# Autodesk Inventor assembly: main
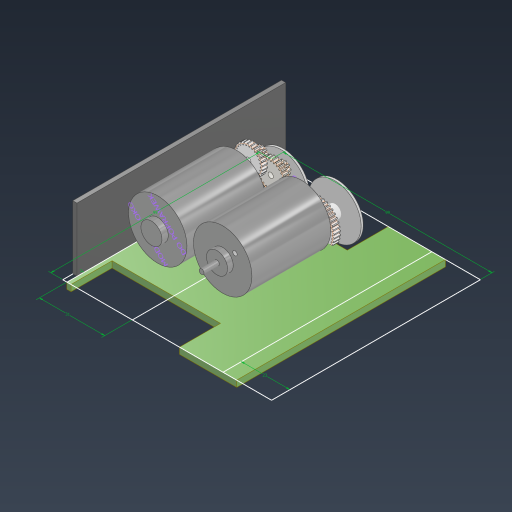
[picture p0: Inventor's stored thumbnail of the model, 512x512]
Saved by Autodesk Inventor 2023 (Build 270158000, 158)
## iProperties
Created: 2025-03-29
Part Number: main
Document SubType Name: Assembly
Designer: szymo
Mass: 421.477 g
Surface Area: 797.238 cm^2
Volume: 148.723 cm^3
Density: 2.83398 g/cm^3
Author: szymo
## Documents named in this file (25)
- D:\tech\robotyka\robots\evangelion\inventor-project\main.iam
- D:\tech\robotyka\robots\evangelion\inventor-project\base.ipt
- D:\tech\robotyka\robots\evangelion\inventor-project\Sensor LUNA.ipt
- D:\tech\robotyka\robots\evangelion\inventor-project\lipo-3s-550mah.ipt
- D:\tech\robotyka\robots\evangelion\inventor-project\tattu450_3s.ipt
- D:\tech\robotyka\robots\evangelion\inventor-project\oponka-dziurawa-prototyp\rs385.ipt
- D:\tech\robotyka\robots\evangelion\inventor-project\oponka-dziurawa-prototyp\back.ipt
- D:\tech\robotyka\robots\evangelion\inventor-project\Gears\Design Accelerator\Przekładnia walcowa14.ipt
- D:\tech\robotyka\robots\evangelion\inventor-project\Gears\Design Accelerator\Przekładnia walcowa22.ipt
- D:\tech\robotyka\robots\evangelion\inventor-project\Gears\Design Accelerator\Przekładnia walcowa23.ipt
- D:\tech\robotyka\robots\evangelion\inventor-project\Gears\Design Accelerator\Przekładnia walcowa24.ipt
- D:\tech\robotyka\robots\evangelion\inventor-project\Gears\Design Accelerator\Przekładnia walcowa12.ipt
- D:\tech\robotyka\robots\evangelion\inventor-project\Gears\Design Accelerator\Przekładnia walcowa13.ipt
- D:\tech\robotyka\robots\evangelion\inventor-project\oponka-dziurawa-prototyp\wheel.ipt
- D:\tech\robotyka\robots\evangelion\inventor-project\Lozysko GFM-0608-2.ipt
- D:\tech\robotyka\robots\evangelion\inventor-project\tattu450_2s.ipt
- D:\tech\robotyka\robots\evangelion\inventor-project\oponka-dziurawa-prototyp\front-mechanizm.iam
- D:\tech\robotyka\robots\evangelion\inventor-project\tfminis\LiDAR Benewake TFMini.iam
- D:\tech\robotyka\robots\evangelion\inventor-project\128x32-OLED.ipt
- D:\tech\robotyka\robots\evangelion\inventor-project\interface_board.ipt
- D:\tech\robotyka\robots\evangelion\inventor-project\front.iam
- D:\tech\robotyka\robots\evangelion\inventor-project\side-right.ipt
- D:\tech\robotyka\robots\evangelion\inventor-project\oponka-dziurawa-prototyp\front-mechanizm_MIR.iam
- D:\tech\robotyka\robots\evangelion\inventor-project\Lozysko GFM-0608-06 very shorted.ipt
- D:\tech\robotyka\robots\evangelion\inventor-project\Lozysko HK0608.ipt
## Components (44 placed, 20 different names)
1. base:1 — Mate:5, Mate:6, Mate:7, Flush:10, Flush:11, Mate:63, Mate:64, Tangent:24, Mate:65, Flush:16, Flush:17, Flush:18, Flush:19, Angle:4, Angle:5, Angle:6, Mate:101, Mate:102, Angle:7
2. rs385:2 — Tangent:6, Mate:53, Mate:54, Tangent:21, Tangent:22, Tangent:23, Mate:101, Tangent:34
3. rs385:3 — Tangent:4, Tangent:5, Mate:102
4. Sensor LUNA:1 — Mate:62, Mate:64, Flush:14
5. Sensor LUNA:2 — Mate:61, Mate:63, Flush:13
6. lipo-3s-550mah:1
7. tattu450_3s:1 — Tangent:21
8. back:1 — Mate:5, Mate:6, Tangent:4, Mate:7, Tangent:5, Tangent:6, Angle:2, Flush:9, Flush:12, Tangent:28, Angle:4
9. tattu450_2s:1 — Flush:9, Mate:58, Tangent:22, Flush:10, Flush:13, Flush:14
10. tattu450_2s:2 — Mate:58, Tangent:23, Mate:61, Mate:62, Flush:11
11. front-mechanizm:1 [sub-assembly] — Tangent:24, Mate:65
12. front-mechanizm_MIR:1 [sub-assembly]
13. front:1 [sub-assembly]
14. side-right:1 — Flush:16, Flush:17, Flush:18, Flush:19
15. LiDAR Benewake TFMini:1 [sub-assembly]
16. LiDAR Benewake TFMini:2 [sub-assembly]
17. 128x32-OLED:1
18. interface_board:1
19. Lozysko HK0608:1 — Mate:91, Mate:93
20. Lozysko HK0608:2 — Mate:92, Mate:94, Tangent:34
21. Przekładnia walcowa2:10 — Tangent:32
22. Przekładnia walcowa1:8 — Mate:99, Mate:100, Tangent:33
23. Przekładnia walcowa1:3
24. Przekładnia walcowa2:1 — Tangent:33
25. Przekładnia walcowa1:2 — Mate:99
26. Przekładnia walcowa1:7 — Tangent:30, Tangent:31
27. Przekładnia walcowa2:9 — Mate:95, Mate:96, Mate:100, Tangent:32
28. Przekładnia walcowa2:4 — Angle:6, Mate:92, Mate:94, Mate:95, Tangent:30, Mate:103, Angle:7
29. Przekładnia walcowa2:3 — Angle:5, Mate:91, Mate:93, Mate:96, Tangent:31, Mate:103
30. wheel:1 — Tangent:29, Flush:20
31. wheel:2 — Tangent:28, Tangent:29, Flush:20
32. Lozysko GFM-0608-06 very shorted:2 — Mate:81, Mate:83
33. Lozysko GFM-0608-06 very shorted:1 — Mate:80, Mate:82
34. Przekładnia walcowa1:4
35. Przekładnia walcowa2:5 — Tangent:17
36. Przekładnia walcowa2:6
37. Przekładnia walcowa2:7 — Mate:55, Angle:3, Mate:80, Mate:82
38. Przekładnia walcowa1:5
39. Przekładnia walcowa1:6 — Mate:53, Mate:54
40. Przekładnia walcowa2:8 — Tangent:17, Mate:55, Mate:81, Mate:83
41. wheel:3 — Tangent:25
42. wheel:4 — Tangent:25
43. Lozysko GFM-0608-2:3
44. Lozysko GFM-0608-2:4
## Relationships (102: Mate 50, Tangent 21, Flush 18, Angle 7, RelateRotation 6)
- [Angle] (0 deg): base:1 ↔ rs385:3
- [Tangent]: rs385:2 ↔ rs385:3
- [Mate]: rs385:3 ↔ Przekładnia walcowa1:3
- [Mate] (0.5 mm): rs385:3 ↔ Przekładnia walcowa1:3
- Mate:5: base:1 ↔ back:1
- Mate:6: base:1 ↔ back:1
- Tangent:4: rs385:3 ↔ back:1
- Mate:7: base:1 ↔ back:1
- Tangent:5: rs385:3 ↔ back:1
- Tangent:6: rs385:2 ↔ back:1
- [Tangent]: Przekładnia walcowa1:3 ↔ Przekładnia walcowa1:2
- [Flush]: Przekładnia walcowa1:3 ↔ Przekładnia walcowa1:2
- [Mate]: Przekładnia walcowa2:1 ↔ Przekładnia walcowa1:2
- [Mate]: Przekładnia walcowa2:1 ↔ Przekładnia walcowa1:2
- [Mate]: Przekładnia walcowa2:4 ↔ wheel:1
- [Flush] (1 mm): Przekładnia walcowa2:4 ↔ wheel:1
- [Mate]: Przekładnia walcowa2:3 ↔ wheel:2
- [Flush] (1 mm): Przekładnia walcowa2:3 ↔ wheel:2
- Angle:2 (0 deg): back:1
- Flush:5 (-49.5 mm)
- [Tangent]: Przekładnia walcowa1:5 ↔ Przekładnia walcowa1:6
- [RelateRotation] (0.4 ul): Przekładnia walcowa1:5 ↔ Przekładnia walcowa1:6
- [Flush]: Przekładnia walcowa1:5 ↔ Przekładnia walcowa1:6
- [Mate]: Przekładnia walcowa2:5 ↔ Przekładnia walcowa1:5
- [Mate]: Przekładnia walcowa2:5 ↔ Przekładnia walcowa1:5
- [RelateRotation] (1 ul): Przekładnia walcowa2:5 ↔ Przekładnia walcowa1:5
- [Mate] (0.1 mm): Przekładnia walcowa2:6 ↔ Przekładnia walcowa1:5
- [Tangent]: Przekładnia walcowa2:5 ↔ Przekładnia walcowa2:6
- [RelateRotation] (0.333 ul): Przekładnia walcowa2:5 ↔ Przekładnia walcowa2:6
- [Mate]: Przekładnia walcowa1:4 ↔ Przekładnia walcowa2:6
- [Mate]: Przekładnia walcowa1:4 ↔ Przekładnia walcowa2:6
- [RelateRotation] (0.5 ul): Przekładnia walcowa1:4 ↔ Przekładnia walcowa2:6
- [Mate] (0.1 mm): Przekładnia walcowa2:6 ↔ Przekładnia walcowa2:7
- [RelateRotation] (0.375 ul): Przekładnia walcowa1:4 ↔ Przekładnia walcowa2:7
- [Mate] (0.1 mm): Przekładnia walcowa2:6 ↔ Przekładnia walcowa2:8
- [Tangent]: Przekładnia walcowa1:4 ↔ Przekładnia walcowa2:8
- [RelateRotation] (2.667 ul): Przekładnia walcowa1:4 ↔ Przekładnia walcowa2:8
- [Mate]: Przekładnia walcowa2:8 ↔ wheel:3
- [Flush] (1 mm): Przekładnia walcowa2:8 ↔ wheel:3
- [Mate]: Przekładnia walcowa2:7 ↔ wheel:4
- [Flush] (1 mm): Przekładnia walcowa2:7 ↔ wheel:4
- [Mate]: Przekładnia walcowa2:7 ↔ Lozysko GFM-0608-2:4
- [Mate]: Przekładnia walcowa2:7 ↔ Lozysko GFM-0608-2:4
- [Mate]: Przekładnia walcowa2:8 ↔ Lozysko GFM-0608-2:3
- [Mate]: Przekładnia walcowa2:8 ↔ Lozysko GFM-0608-2:3
- Mate:53 (0.5 mm): rs385:2 ↔ Przekładnia walcowa1:6
- Mate:54: rs385:2 ↔ Przekładnia walcowa1:6
- Tangent:17 (0.5 mm): Przekładnia walcowa2:5 ↔ Przekładnia walcowa2:8
- Mate:55: Przekładnia walcowa2:7 ↔ Przekładnia walcowa2:8
- Angle:3 (0 deg): Przekładnia walcowa2:7
- Tangent:21 (1 mm): rs385:2 ↔ tattu450_3s:1
- Flush:9: back:1 ↔ tattu450_2s:1
- Mate:58: tattu450_2s:1 ↔ tattu450_2s:2
- Tangent:22: rs385:2 ↔ tattu450_2s:1
- Tangent:23: rs385:2 ↔ tattu450_2s:2
- Mate:61: Sensor LUNA:2 ↔ tattu450_2s:2
- Mate:62: Sensor LUNA:1 ↔ tattu450_2s:2
- Flush:10 (15.5 mm): base:1 ↔ tattu450_2s:1
- Flush:11 (15.5 mm): base:1 ↔ tattu450_2s:2
- Mate:63 (1.5 mm): base:1 ↔ Sensor LUNA:2
- Mate:64 (1.5 mm): base:1 ↔ Sensor LUNA:1
- Flush:12 (87 mm): back:1
- Tangent:24 (3.5 mm): base:1 ↔ front-mechanizm:1
- Mate:65: base:1 ↔ front-mechanizm:1
- Flush:13: Sensor LUNA:2 ↔ tattu450_2s:1
- Flush:14: Sensor LUNA:1 ↔ tattu450_2s:1
- Tangent:25 (1 mm): wheel:3 ↔ wheel:4
- Flush:16: base:1 ↔ side-right:1
- Flush:17: base:1 ↔ side-right:1
- Flush:18: base:1 ↔ side-right:1
- Flush:19: base:1 ↔ side-right:1
- Mate:80 (0.1 mm): Lozysko GFM-0608-06 very shorted:1 ↔ Przekładnia walcowa2:7
- Mate:81 (0.1 mm): Lozysko GFM-0608-06 very shorted:2 ↔ Przekładnia walcowa2:8
- Mate:82: Lozysko GFM-0608-06 very shorted:1 ↔ Przekładnia walcowa2:7
- Mate:83: Lozysko GFM-0608-06 very shorted:2 ↔ Przekładnia walcowa2:8
- [Mate]: Przekładnia walcowa1:7 ↔ Przekładnia walcowa2:9
- [Mate]: Przekładnia walcowa1:7 ↔ Przekładnia walcowa2:9
- Tangent:28 (0.5 mm): back:1 ↔ wheel:2
- Angle:4 (-90 deg): base:1 ↔ back:1
- Tangent:29 (0.5 mm): wheel:1 ↔ wheel:2
- Angle:5 (180 deg): base:1 ↔ Przekładnia walcowa2:3
- Angle:6 (180 deg): base:1 ↔ Przekładnia walcowa2:4
- Flush:20: wheel:1 ↔ wheel:2
- Mate:91: Lozysko HK0608:1 ↔ Przekładnia walcowa2:3
- Mate:92: Lozysko HK0608:2 ↔ Przekładnia walcowa2:4
- Mate:93 (0.1 mm): Lozysko HK0608:1 ↔ Przekładnia walcowa2:3
- Mate:94 (0.1 mm): Lozysko HK0608:2 ↔ Przekładnia walcowa2:4
- Mate:95 (0.1 mm): Przekładnia walcowa2:9 ↔ Przekładnia walcowa2:4
- Mate:96 (0.1 mm): Przekładnia walcowa2:9 ↔ Przekładnia walcowa2:3
- Tangent:30: Przekładnia walcowa1:7 ↔ Przekładnia walcowa2:4
- Tangent:31: Przekładnia walcowa1:7 ↔ Przekładnia walcowa2:3
- [Mate]: Przekładnia walcowa2:10 ↔ Przekładnia walcowa1:8
- [Mate]: Przekładnia walcowa2:10 ↔ Przekładnia walcowa1:8
- Mate:99 (0.1 mm): Przekładnia walcowa1:8 ↔ Przekładnia walcowa1:2
- Mate:100 (0.1 mm): Przekładnia walcowa1:8 ↔ Przekładnia walcowa2:9
- Tangent:32: Przekładnia walcowa2:10 ↔ Przekładnia walcowa2:9
- Tangent:33: Przekładnia walcowa1:8 ↔ Przekładnia walcowa2:1
- Mate:101 (29.65 mm): base:1 ↔ rs385:2
- Mate:102 (29.65 mm): base:1 ↔ rs385:3
- Mate:103: Przekładnia walcowa2:4 ↔ Przekładnia walcowa2:3
- Angle:7 (0 deg): base:1 ↔ Przekładnia walcowa2:4
- Tangent:34 (0.2 mm): rs385:2 ↔ Lozysko HK0608:2
## Named parameters: d53_d28 = 0 mm, d54_d29 = 0 mm, d208_d31 = 0.1 mm, d209_d32 = 0 mm, d210_d58_d33 = 0.333, d211_d59_d34 = 0 mm, d212_d60_d35 = 0 mm, d213_d61_d36 = 0.5, d214_d62_d37 = 0.1 mm, d216_d64_d39 = 0.375, d217_d67 = 1 mm, d218_d61 = 0.1 mm, d219_d62 = 0 mm, d220_d63 = 2.667, d221_d64 = 0 mm, d222_d65 = 1 mm, d223_d66 = 0 mm, d230_d88 = 0 mm, d231_d89 = 0 mm, d232_d90 = 0 mm, d233_d91 = 0 mm, d234_d25 = 0 mm, d235_d26 = 0.4, d236_d27 = 0 mm, d237_d53_d28 = 0 mm, d238_d54_d29 = 0 mm, d239_d30 = 1, d333_d59_d34 = 0 mm, d334_d60_d35 = 0 mm, d357_d53_d28 = 0 mm, d358_d54_d29 = 0 mm
